# Autodesk Inventor assembly: 00_004_FEMUR_R1
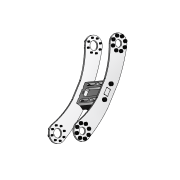
[picture p0: Inventor's stored thumbnail of the model, 180x180]
Saved by Autodesk Inventor 2021.2 (Build 252289000, 289)
## iProperties
Created: 2021-01-16
Part Number: 00_004_FEMUR_R1
Document SubType Name: Assembly
Designer: y6tada
Author: y6tada
## Documents named in this file (8)
- C:\Workspace\HaptHexa\Hardware\Inventor\00_004_FEMUR_R1.iam
- C:\Workspace\HaptHexa\Hardware\Inventor\16_013_FEMUR_FRAME_FREE_R1.ipt
- C:\Workspace\HaptHexa\Hardware\Inventor\16_012_FEMUR_FRAME_DRIVER_R1.ipt
- C:\Workspace\HaptHexa\Hardware\Inventor\16_010_FEMUR_BRIDGE_R1.ipt
- C:\Workspace\HaptHexa\Hardware\Inventor\15_011_FEMUR_BRIDGE_SUPPORT_R1.ipt
- C:\Workspace\HaptHexa\Hardware\Inventor\10_054_CAP_BOLT_M2_5X8_R1.ipt
- C:\Workspace\HaptHexa\Hardware\Inventor\10_051_LOW_HEAD_CAP_BOLT_M3X6_R1.ipt
- C:\Workspace\HaptHexa\Hardware\Inventor\10_048_CAP_SCREW_M2X4_R1.ipt
## Components (42 placed, 7 different names)
1. 16_013_FEMUR_FRAME_FREE_R1:1 — Insert:7, Insert:8
2. 16_012_FEMUR_FRAME_DRIVER_R1:1 — Insert:3, Insert:4
3. 16_010_FEMUR_BRIDGE_R1:1
4. 15_011_FEMUR_BRIDGE_SUPPORT_R1:1 — Insert:5, Insert:6
5. 10_054_CAP_BOLT_M2_5X8_R1:1 — Insert:3
6. 10_054_CAP_BOLT_M2_5X8_R1:2 — Insert:4
7. 10_051_LOW_HEAD_CAP_BOLT_M3X6_R1:1 — Insert:5
8. 10_054_CAP_BOLT_M2_5X8_R1:3 — Insert:8
9. 10_054_CAP_BOLT_M2_5X8_R1:4 — Insert:7
10. 10_051_LOW_HEAD_CAP_BOLT_M3X6_R1:2 — Insert:6
11. 10_048_CAP_SCREW_M2X4_R1:3
12. 10_048_CAP_SCREW_M2X4_R1:1
13. 10_048_CAP_SCREW_M2X4_R1:5
14. 10_048_CAP_SCREW_M2X4_R1:6
15. 10_048_CAP_SCREW_M2X4_R1:7
16. 10_048_CAP_SCREW_M2X4_R1:8
17. 10_048_CAP_SCREW_M2X4_R1:9
18. 10_048_CAP_SCREW_M2X4_R1:10
19. 10_048_CAP_SCREW_M2X4_R1:11
20. 10_048_CAP_SCREW_M2X4_R1:12
21. 10_048_CAP_SCREW_M2X4_R1:13
22. 10_048_CAP_SCREW_M2X4_R1:14
23. 10_048_CAP_SCREW_M2X4_R1:15
24. 10_048_CAP_SCREW_M2X4_R1:16
25. 10_048_CAP_SCREW_M2X4_R1:17
26. 10_048_CAP_SCREW_M2X4_R1:18
27. 10_048_CAP_SCREW_M2X4_R1:2
28. 10_048_CAP_SCREW_M2X4_R1:4
29. 10_048_CAP_SCREW_M2X4_R1:19
30. 10_048_CAP_SCREW_M2X4_R1:20
31. 10_048_CAP_SCREW_M2X4_R1:21
32. 10_048_CAP_SCREW_M2X4_R1:22
33. 10_048_CAP_SCREW_M2X4_R1:23
34. 10_048_CAP_SCREW_M2X4_R1:24
35. 10_048_CAP_SCREW_M2X4_R1:25
36. 10_048_CAP_SCREW_M2X4_R1:26
37. 10_048_CAP_SCREW_M2X4_R1:27
38. 10_048_CAP_SCREW_M2X4_R1:28
39. 10_048_CAP_SCREW_M2X4_R1:29
40. 10_048_CAP_SCREW_M2X4_R1:30
41. 10_048_CAP_SCREW_M2X4_R1:31
42. 10_048_CAP_SCREW_M2X4_R1:32
## Component patterns: (8 elements, first: 10_048_CAP_SCREW_M2X4_R1:3 + 10_048_CAP_SCREW_M2X4_R1:1), (8 elements, first: 10_048_CAP_SCREW_M2X4_R1:2 + 10_048_CAP_SCREW_M2X4_R1:4)
## Relationships (17: Insert 12, Mate 4, Flush 1)
- [Insert]: 16_013_FEMUR_FRAME_FREE_R1:1 ↔ 16_010_FEMUR_BRIDGE_R1:1
- [Insert]: 16_012_FEMUR_FRAME_DRIVER_R1:1 ↔ 16_010_FEMUR_BRIDGE_R1:1
- [Mate]: 16_012_FEMUR_FRAME_DRIVER_R1:1 ↔ 16_010_FEMUR_BRIDGE_R1:1
- [Mate]: 16_013_FEMUR_FRAME_FREE_R1:1 ↔ 16_010_FEMUR_BRIDGE_R1:1
- [Flush]: 16_010_FEMUR_BRIDGE_R1:1 ↔ 15_011_FEMUR_BRIDGE_SUPPORT_R1:1
- [Mate]: 16_010_FEMUR_BRIDGE_R1:1 ↔ 15_011_FEMUR_BRIDGE_SUPPORT_R1:1
- [Mate]: 16_010_FEMUR_BRIDGE_R1:1 ↔ 15_011_FEMUR_BRIDGE_SUPPORT_R1:1
- Insert:3: 16_012_FEMUR_FRAME_DRIVER_R1:1 ↔ 10_054_CAP_BOLT_M2_5X8_R1:1
- Insert:4: 16_012_FEMUR_FRAME_DRIVER_R1:1 ↔ 10_054_CAP_BOLT_M2_5X8_R1:2
- Insert:5: 15_011_FEMUR_BRIDGE_SUPPORT_R1:1 ↔ 10_051_LOW_HEAD_CAP_BOLT_M3X6_R1:1
- Insert:6: 15_011_FEMUR_BRIDGE_SUPPORT_R1:1 ↔ 10_051_LOW_HEAD_CAP_BOLT_M3X6_R1:2
- Insert:7: 16_013_FEMUR_FRAME_FREE_R1:1 ↔ 10_054_CAP_BOLT_M2_5X8_R1:4
- Insert:8: 16_013_FEMUR_FRAME_FREE_R1:1 ↔ 10_054_CAP_BOLT_M2_5X8_R1:3
- [Insert]: 16_013_FEMUR_FRAME_FREE_R1:1 ↔ 10_048_CAP_SCREW_M2X4_R1:1
- [Insert]: 16_012_FEMUR_FRAME_DRIVER_R1:1 ↔ 10_048_CAP_SCREW_M2X4_R1:2
- [Insert]: 16_012_FEMUR_FRAME_DRIVER_R1:1 ↔ 10_048_CAP_SCREW_M2X4_R1:3
- [Insert]: 16_013_FEMUR_FRAME_FREE_R1:1 ↔ 10_048_CAP_SCREW_M2X4_R1:4
